# Autodesk Inventor assembly: linkage_system_v-upper
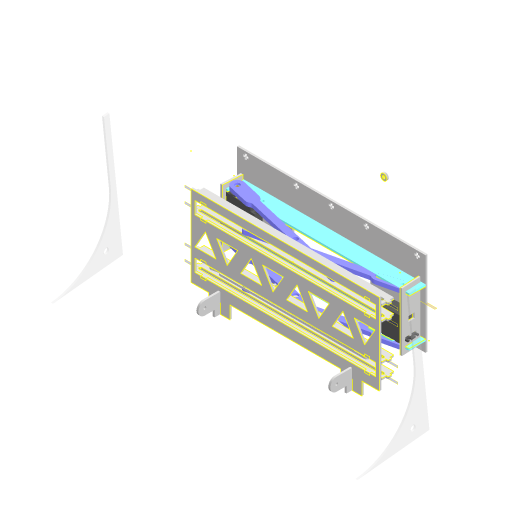
[picture p0: Inventor's stored thumbnail of the model, 512x512]
Saved by Autodesk Inventor 2023 (Build 270158000, 158)
## iProperties
Created: 2023-05-05
Part Number: linkage_system_v-upper
Document SubType Name: Assembly
Designer: 陳詩穎
Author: 陳詩穎
## Documents named in this file (18)
- D:\Areo_Rider_Cabin\Expansion\test\linkage_system_v-upper.iam
- D:\Areo_Rider_Cabin\Expansion\test\plate_expansion.ipt
- D:\Areo_Rider_Cabin\Expansion\test\零件1.ipt
- D:\Areo_Rider_Cabin\Expansion\test\零件4.ipt
- D:\Areo_Rider_Cabin\Expansion\test\零件5.ipt
- D:\Areo_Rider_Cabin\Expansion\test\零件7.ipt
- D:\Areo_Rider_Cabin\Airfoil & Nuzzle\nuzzle\nuzzle_v2_0327.ipt
- D:\Areo_Rider_Cabin\Airfoil & Nuzzle\nuzzle\nuzzle_v2_0516.ipt
- D:\Areo_Rider_Cabin\Airfoil & Nuzzle\nuzzle\nuzzle_v2_0516_2.ipt
- D:\Areo_Rider_Cabin\Expansion\test\零件8.ipt
- D:\Areo_Rider_Cabin\Expansion\test\零件9.ipt
- D:\Areo_Rider_Cabin\Expansion\test\零件10.ipt
- D:\Areo_Rider_Cabin\Expansion\test\零件12.ipt
- D:\Areo_Rider_Cabin\Expansion\test\adjustable_130.ipt
- D:\Areo_Rider_Cabin\Expansion\test\adjustable_80.ipt
- D:\Areo_Rider_Cabin\Expansion\test\零件13.ipt
- D:\Areo_Rider_Cabin\car\外抓檔\Tower Pro MG996R.ipt
- D:\Areo_Rider_Cabin\Expansion\test\200_forservo.ipt
## Components (30 placed, 17 different names)
1. plate_expansion:1 — 貼合:1, 齊平:1, 貼合:2, 角度:1, 齊平:13, 貼合:255, 齊平:27
2. 零件1:2 — 貼合:1, 齊平:1, 貼合:2, 貼合:49, 貼合:51, 貼合:226, 插入:32, 齊平:28, 貼合:260, 插入:57
3. 零件8:1 — 貼合:49, 貼合:51, 貼合:258
4. 零件4:1 — 齊平:8, 齊平:9, 齊平:10, 貼合:187, 貼合:261, 相切:5, 相切:6
5. 零件4:2 — 齊平:7, 齊平:8, 貼合:189, 貼合:262, 相切:2
6. 零件4:3 — 齊平:9, 貼合:188, 貼合:191, 相切:3, 相切:4
7. 零件4:4 — 齊平:7, 貼合:190, 貼合:263, 貼合:274, 相切:1
8. 零件5:1 — 齊平:10, 貼合:187, 貼合:188, 貼合:189, 貼合:190, 貼合:191, 角度:1, 齊平:13, 齊平:17, 貼合:208, 貼合:209, 貼合:210, 貼合:211, 貼合:212, 貼合:213, 貼合:261, 貼合:262, 貼合:263
9. nuzzle_v2_0327:1 — 齊平:17, 貼合:200, 貼合:201
10. nuzzle_v2_0516:1 — 貼合:202, 貼合:203, 貼合:204, 貼合:205, 齊平:18
11. nuzzle_v2_0516_2:1 — 貼合:200, 貼合:201, 貼合:202, 貼合:203, 貼合:206, 齊平:19
12. 零件9:1 — 貼合:204, 貼合:205, 貼合:207, 齊平:18
13. 零件10:1 — 貼合:206, 貼合:207, 齊平:19, 貼合:214
14. 零件7:1 — 貼合:208, 貼合:209, 貼合:210, 貼合:214
15. 零件7:2 — 貼合:211, 貼合:212, 貼合:213
16. 零件8:2 — 貼合:226, 貼合:259, 貼合:260
17. Tower Pro MG996R:1 — 插入:33, 貼合:258, 插入:60
18. Tower Pro MG996R:2 — 插入:32, 貼合:259, 插入:56
19. 零件1:3 — 貼合:255, 齊平:27, 齊平:28, 插入:33, 插入:63
20. adjustable_130:1 — 插入:54, 插入:61
21. 零件12:2 — 插入:55, 插入:62
22. adjustable_80:2 — 相切:4
23. adjustable_130:2 — 插入:58
24. 零件12:3 — 插入:59
25. adjustable_80:3 — 插入:54, 插入:55, 相切:6
26. 200_forservo:1 — 插入:56, 貼合:274, 相切:1
27. 200_forservo:2 — 插入:58, 插入:59, 插入:60, 相切:3
28. 200_forservo:3 — 插入:61, 插入:62, 插入:63, 相切:5
29. 200_forservo:4 — 插入:57, 相切:2
30. 零件13:2
## Relationships (65: Mate 33, Insert 14, Flush 11, Tangent 6, Angle 1)
- 貼合:1 [Mate]: plate_expansion:1 ↔ 零件1:2
- 齊平:1 [Flush]: plate_expansion:1 ↔ 零件1:2
- 貼合:2 [Mate]: plate_expansion:1 ↔ 零件1:2
- 貼合:49 [Mate]: 零件1:2 ↔ 零件8:1
- 貼合:51 [Mate]: 零件1:2 ↔ 零件8:1
- 齊平:7 [Flush]: 零件4:2 ↔ 零件4:4
- 齊平:8 [Flush]: 零件4:1 ↔ 零件4:2
- 齊平:9 [Flush]: 零件4:1 ↔ 零件4:3
- 齊平:10 [Flush]: 零件4:1 ↔ 零件5:1
- 貼合:187 [Mate]: 零件4:1 ↔ 零件5:1
- 貼合:188 [Mate]: 零件4:3 ↔ 零件5:1
- 貼合:189 [Mate]: 零件4:2 ↔ 零件5:1
- 貼合:190 [Mate]: 零件4:4 ↔ 零件5:1
- 貼合:191 [Mate]: 零件4:3 ↔ 零件5:1
- 角度:1 [Angle] (0 deg): plate_expansion:1 ↔ 零件5:1
- 齊平:13 [Flush]: plate_expansion:1 ↔ 零件5:1
- 齊平:17 [Flush] (-2 mm): 零件5:1 ↔ nuzzle_v2_0327:1
- 貼合:200 [Mate]: nuzzle_v2_0327:1 ↔ nuzzle_v2_0516_2:1
- 貼合:201 [Mate]: nuzzle_v2_0327:1 ↔ nuzzle_v2_0516_2:1
- 貼合:202 [Mate]: nuzzle_v2_0516:1 ↔ nuzzle_v2_0516_2:1
- 貼合:203 [Mate]: nuzzle_v2_0516:1 ↔ nuzzle_v2_0516_2:1
- 貼合:204 [Mate]: nuzzle_v2_0516:1 ↔ 零件9:1
- 貼合:205 [Mate]: nuzzle_v2_0516:1 ↔ 零件9:1
- 貼合:206 [Mate]: nuzzle_v2_0516_2:1 ↔ 零件10:1
- 貼合:207 [Mate]: 零件9:1 ↔ 零件10:1
- 齊平:18 [Flush] (-20 mm): nuzzle_v2_0516:1 ↔ 零件9:1
- 齊平:19 [Flush] (20 mm): nuzzle_v2_0516_2:1 ↔ 零件10:1
- 貼合:208 [Mate]: 零件5:1 ↔ 零件7:1
- 貼合:209 [Mate]: 零件5:1 ↔ 零件7:1
- 貼合:210 [Mate]: 零件5:1 ↔ 零件7:1
- 貼合:211 [Mate]: 零件5:1 ↔ 零件7:2
- 貼合:212 [Mate]: 零件5:1 ↔ 零件7:2
- 貼合:213 [Mate]: 零件5:1 ↔ 零件7:2
- 貼合:214 [Mate]: 零件10:1 ↔ 零件7:1
- 貼合:226 [Mate]: 零件1:2 ↔ 零件8:2
- 插入:32 [Insert]: 零件1:2 ↔ Tower Pro MG996R:2
- 貼合:255 [Mate]: plate_expansion:1 ↔ 零件1:3
- 齊平:27 [Flush]: plate_expansion:1 ↔ 零件1:3
- 齊平:28 [Flush]: 零件1:2 ↔ 零件1:3
- 插入:33 [Insert]: Tower Pro MG996R:1 ↔ 零件1:3
- 貼合:258 [Mate]: 零件8:1 ↔ Tower Pro MG996R:1
- 貼合:259 [Mate]: 零件8:2 ↔ Tower Pro MG996R:2
- 貼合:260 [Mate]: 零件1:2 ↔ 零件8:2
- 貼合:261 [Mate]: 零件4:1 ↔ 零件5:1
- 貼合:262 [Mate]: 零件4:2 ↔ 零件5:1
- 貼合:263 [Mate]: 零件4:4 ↔ 零件5:1
- [Insert]: adjustable_80:2 ↔ 零件12:3
- [Insert]: adjustable_80:2 ↔ adjustable_130:2
- 插入:54 [Insert]: adjustable_130:1 ↔ adjustable_80:3
- 插入:55 [Insert]: 零件12:2 ↔ adjustable_80:3
- 插入:56 [Insert]: Tower Pro MG996R:2 ↔ 200_forservo:1
- 貼合:274 [Mate]: 零件4:4 ↔ 200_forservo:1
- 相切:1 [Tangent]: 零件4:4 ↔ 200_forservo:1
- 插入:57 [Insert]: 零件1:2 ↔ 200_forservo:4
- 相切:2 [Tangent]: 零件4:2 ↔ 200_forservo:4
- 插入:58 [Insert]: adjustable_130:2 ↔ 200_forservo:2
- 插入:59 [Insert]: 零件12:3 ↔ 200_forservo:2
- 插入:60 [Insert]: Tower Pro MG996R:1 ↔ 200_forservo:2
- 相切:3 [Tangent]: 零件4:3 ↔ 200_forservo:2
- 相切:4 [Tangent]: 零件4:3 ↔ adjustable_80:2
- 插入:61 [Insert]: adjustable_130:1 ↔ 200_forservo:3
- 插入:62 [Insert]: 零件12:2 ↔ 200_forservo:3
- 插入:63 [Insert]: 零件1:3 ↔ 200_forservo:3
- 相切:5 [Tangent]: 零件4:1 ↔ 200_forservo:3
- 相切:6 [Tangent]: 零件4:1 ↔ adjustable_80:3
## Named parameters: d455_d451 = 0 mm, d456_d452 = 0 mm
